# Autodesk Inventor assembly: Switch D3SH-A1R1
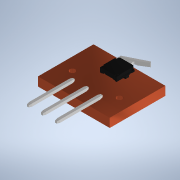
[picture p0: Inventor's stored thumbnail of the model, 180x180]
Saved by Autodesk Inventor 2020.3 (Build 243373000, 373)
## iProperties
Created: 2020-06-27
Part Number: Switch D3SH-A1R1
Document SubType Name: Assembly
Designer: javic
Author: javic
## Documents named in this file (4)
- C:\Users\javic\Downloads\Universidad\2020-1\Seminario - SPEL\InterStage\Componentes\Piezas\Switch D3SH-A1R1.iam
- C:\Users\javic\Downloads\Universidad\2020-1\Seminario - SPEL\InterStage\Componentes\Piezas\Placa Cobre.ipt
- C:\Users\javic\Downloads\Universidad\2020-1\Seminario - SPEL\InterStage\Componentes\Piezas\Switch D3SH-A1R1.ipt
- C:\Users\javic\Downloads\Universidad\2020-1\Seminario - SPEL\InterStage\Componentes\Piezas\Conector 3 pines.ipt
## Components (3 placed, 3 different names)
1. Placa Cobre:1 — Coincidencia:1, Coincidencia:2, Nivelación:1, Coincidencia:3, Nivelación:2, Nivelación:3
2. Switch D3SH-A1R1:1 — Coincidencia:1, Coincidencia:2, Nivelación:1
3. Conector 3 pines:1 — Coincidencia:3, Nivelación:2, Nivelación:3
## Relationships (6: Mate 3, Flush 3)
- Coincidencia:1 [Mate]: Placa Cobre:1 ↔ Switch D3SH-A1R1:1
- Coincidencia:2 [Mate] (-3.8 mm): Placa Cobre:1 ↔ Switch D3SH-A1R1:1
- Nivelación:1 [Flush] (5 mm): Placa Cobre:1 ↔ Switch D3SH-A1R1:1
- Coincidencia:3 [Mate]: Placa Cobre:1 ↔ Conector 3 pines:1
- Nivelación:2 [Flush] (3.71 mm): Placa Cobre:1 ↔ Conector 3 pines:1
- Nivelación:3 [Flush] (7.56 mm): Placa Cobre:1 ↔ Conector 3 pines:1
